# Autodesk Inventor assembly: Existing_Attic
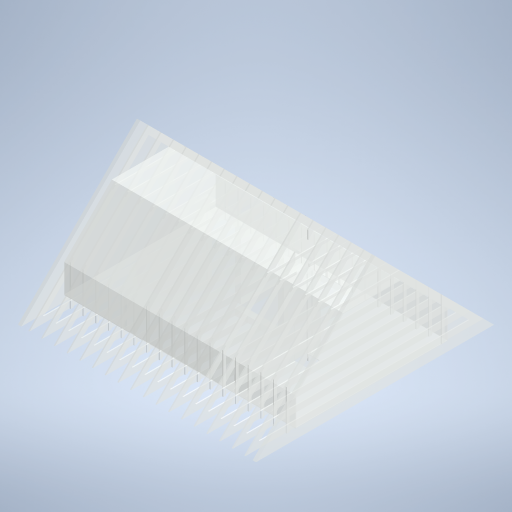
[picture p0: Inventor's stored thumbnail of the model, 512x512]
Saved by Autodesk Inventor 2024 (Build 280153000, 153)
## iProperties
Created: 2023-05-19
Part Number: Existing_Attic
Document SubType Name: Assembly
Designer: Tom
Author: Tom
## Documents named in this file (17)
- C:\Users\Tom\Documents\Tom_Levers_Public_Git_Repository\Inventor\Mobility\Attic\Existing_Attic.iam
- C:\Users\Tom\Documents\Tom_Levers_Public_Git_Repository\Inventor\Mobility\Attic\Gable.ipt
- C:\Users\Tom\Documents\Tom_Levers_Public_Git_Repository\Inventor\Mobility\Attic\Truss.ipt
- C:\Users\Tom\Documents\Tom_Levers_Public_Git_Repository\Inventor\Mobility\Attic\Sheathing.ipt
- C:\Users\Tom\Documents\Tom_Levers_Public_Git_Repository\Inventor\Mobility\Attic\Beam--7.5_x_7.5_x_46.5.ipt
- C:\Users\Tom\Documents\Tom_Levers_Public_Git_Repository\Inventor\Mobility\Attic\Second_Subfloor.ipt
- C:\Users\Tom\Documents\Tom_Levers_Public_Git_Repository\Inventor\Mobility\Attic\Knee_Wall.ipt
- C:\Users\Tom\Documents\Tom_Levers_Public_Git_Repository\Inventor\Mobility\Attic\Second_Ceiling.ipt
- C:\Users\Tom\Documents\Tom_Levers_Public_Git_Repository\Inventor\Mobility\Attic\Drywall_On_Rafters.ipt
- C:\Users\Tom\Documents\Tom_Levers_Public_Git_Repository\Inventor\Mobility\Attic\Wall_Between_Attic_Room_And_Stairwell.ipt
- C:\Users\Tom\Documents\Tom_Levers_Public_Git_Repository\Inventor\Mobility\Attic\Wall_With_Door_For_Attic_Room.ipt
- C:\Users\Tom\Documents\Tom_Levers_Public_Git_Repository\Inventor\Mobility\Attic\Wall_Between_Attic_Room_And_Landing.ipt
- C:\Users\Tom\Documents\Tom_Levers_Public_Git_Repository\Inventor\Mobility\Attic\Tar_Paper.ipt
- C:\Users\Tom\Documents\Tom_Levers_Public_Git_Repository\Inventor\Mobility\Attic\Shingles_On_Tar_Paper.ipt
- C:\Users\Tom\Documents\Tom_Levers_Public_Git_Repository\Inventor\Mobility\Attic\Ridge_Vent.ipt
- C:\Users\Tom\Documents\Tom_Levers_Public_Git_Repository\Inventor\Mobility\Attic\Shingles_On_Ridge_Vent.ipt
- C:\Users\Tom\Documents\Tom_Levers_Public_Git_Repository\Inventor\Mobility\Attic\Drywall.ipt
## Components (43 placed, 16 different names)
1. Gable:1 — Flush:1, Flush:2, Mate:1, Flush:3, Flush:4, Flush:14, Flush:15, Mate:22, Mate:47
2. Gable:2 — Flush:1, Flush:2, Mate:1, Mate:3, Flush:5, Flush:6, Flush:7, Mate:4, Flush:8, Mate:10
3. Sheathing:1 — Mate:3, Flush:5, Flush:6, Flush:23, Mate:39, Flush:24, Flush:26, Flush:29
4. Sheathing:2 — Flush:7, Mate:4, Flush:8, Mate:38, Flush:22, Flush:25, Flush:27, Flush:28, Flush:30
5. Beam--7.5_x_7.5_x_46.5:1 — Mate:5, Flush:9, Mate:6
6. Beam--7.5_x_7.5_x_46.5:2 — Flush:10, Mate:8, Mate:9
7. Second_Subfloor:1 — Mate:10, Mate:11, Mate:12, Flush:11, Mate:13, Flush:12, Mate:15, Flush:13, Mate:25, Flush:18, Mate:27, Flush:19, Mate:29, Mate:31, Mate:32, Mate:35, Mate:49
8. Knee_Wall:1 — Flush:11, Mate:13, Mate:14, Mate:19, Mate:33, Mate:36
9. Knee_Wall:2 — Flush:12, Mate:15, Mate:16, Mate:24, Mate:26
10. Second_Ceiling:1 — Mate:17, Flush:13, Flush:15, Flush:16, Flush:17, Mate:23
11. Drywall_On_Rafters:1 — Flush:16, Mate:18, Mate:19
12. Drywall_On_Rafters:2 — Flush:17, Mate:21, Mate:23
13. Drywall:1 — Mate:47, Mate:48, Mate:49
14. Wall_Between_Attic_Room_And_Stairwell:1 — Mate:24, Mate:25, Flush:18, Mate:30, Flush:21
15. Wall_Between_Attic_Room_And_Stairwell:2 — Mate:26, Mate:27, Flush:19, Mate:28, Flush:20
16. Wall_With_Door_For_Attic_Room:1 — Mate:28, Flush:20, Mate:29, Mate:50
17. Wall_With_Door_For_Attic_Room:2 — Mate:30, Flush:21, Mate:31, Mate:37
18. Wall_Between_Attic_Room_And_Landing:1 — Mate:32, Mate:33, Mate:50
19. Wall_Between_Attic_Room_And_Landing:2 — Mate:35, Mate:36, Mate:37
20. Tar_Paper:1 — Mate:38, Flush:22, Flush:23, Mate:41
21. Tar_Paper:2 — Mate:39, Flush:24, Flush:25, Mate:40
22. Shingles_On_Tar_Paper:1 — Mate:40, Flush:26, Flush:27, Mate:42
23. Shingles_On_Tar_Paper:2 — Mate:41, Flush:28, Flush:29, Mate:43
24. Ridge_Vent:1 — Mate:42, Mate:43, Flush:30, Mate:44, Mate:45, Flush:31
25. Shingles_On_Ridge_Vent:1 — Mate:44, Mate:45, Flush:31
26. Truss:1 — Flush:3, Flush:4, Mate:22
27. Truss:2 — Mate:12
28. Truss:3
29. Truss:4
30. Truss:5 — Mate:11
31. Truss:6
32. Truss:7
33. Truss:8 — Mate:6, Mate:8
34. Truss:9
35. Truss:10 — Mate:5, Flush:9, Flush:10
36. Truss:11 — Mate:9
37. Truss:12
38. Truss:13
39. Truss:14
40. Truss:15
41. Truss:16
42. Truss:17
43. Truss:18 — Mate:14, Mate:16, Mate:17, Mate:18, Mate:20, Mate:21, Mate:48
## Component patterns: (18 elements, first: Truss:1)
## Relationships (77: Mate 46, Flush 31)
- Flush:1: Gable:1 ↔ Gable:2
- Flush:2: Gable:1 ↔ Gable:2
- Mate:1 (7404.1 mm): Gable:1 ↔ Gable:2
- Flush:3: Gable:1 ↔ Truss:1
- Flush:4: Gable:1 ↔ Truss:1
- Mate:3: Gable:2 ↔ Sheathing:1
- Flush:5 (88.9 mm): Gable:2 ↔ Sheathing:1
- Flush:6: Gable:2 ↔ Sheathing:1
- Flush:7 (88.9 mm): Gable:2 ↔ Sheathing:2
- Mate:4: Gable:2 ↔ Sheathing:2
- Flush:8: Gable:2 ↔ Sheathing:2
- Mate:5: Beam--7.5_x_7.5_x_46.5:1 ↔ Truss:10
- Flush:9: Beam--7.5_x_7.5_x_46.5:1 ↔ Truss:10
- Mate:6: Beam--7.5_x_7.5_x_46.5:1 ↔ Truss:8
- Flush:10: Beam--7.5_x_7.5_x_46.5:2 ↔ Truss:10
- Mate:8: Beam--7.5_x_7.5_x_46.5:2 ↔ Truss:8
- Mate:9: Beam--7.5_x_7.5_x_46.5:2 ↔ Truss:11
- Mate:10: Gable:2 ↔ Second_Subfloor:1
- Mate:11: Second_Subfloor:1 ↔ Truss:5
- Mate:12: Second_Subfloor:1 ↔ Truss:2
- Flush:11: Second_Subfloor:1 ↔ Knee_Wall:1
- Mate:13: Second_Subfloor:1 ↔ Knee_Wall:1
- Mate:14: Knee_Wall:1 ↔ Truss:18
- Flush:12: Second_Subfloor:1 ↔ Knee_Wall:2
- Mate:15: Second_Subfloor:1 ↔ Knee_Wall:2
- Mate:16: Knee_Wall:2 ↔ Truss:18
- Mate:17: Second_Ceiling:1 ↔ Truss:18
- Flush:13: Second_Subfloor:1 ↔ Second_Ceiling:1
- Flush:14: Gable:1
- Flush:15: Gable:1 ↔ Second_Ceiling:1
- Flush:16: Second_Ceiling:1 ↔ Drywall_On_Rafters:1
- Mate:18: Drywall_On_Rafters:1 ↔ Truss:18
- Mate:19: Knee_Wall:1 ↔ Drywall_On_Rafters:1
- Mate:20: Truss:18
- Flush:17: Second_Ceiling:1 ↔ Drywall_On_Rafters:2
- Mate:21: Drywall_On_Rafters:2 ↔ Truss:18
- Mate:22 (228.6 mm): Gable:1 ↔ Truss:1
- Mate:23: Second_Ceiling:1 ↔ Drywall_On_Rafters:2
- Mate:24: Knee_Wall:2 ↔ Wall_Between_Attic_Room_And_Stairwell:1
- Mate:25: Second_Subfloor:1 ↔ Wall_Between_Attic_Room_And_Stairwell:1
- Flush:18 (4292.6 mm): Second_Subfloor:1 ↔ Wall_Between_Attic_Room_And_Stairwell:1
- Mate:26: Knee_Wall:2 ↔ Wall_Between_Attic_Room_And_Stairwell:2
- Mate:27: Second_Subfloor:1 ↔ Wall_Between_Attic_Room_And_Stairwell:2
- Flush:19 (2984.5 mm): Second_Subfloor:1 ↔ Wall_Between_Attic_Room_And_Stairwell:2
- Mate:28: Wall_Between_Attic_Room_And_Stairwell:2 ↔ Wall_With_Door_For_Attic_Room:1
- Flush:20: Wall_Between_Attic_Room_And_Stairwell:2 ↔ Wall_With_Door_For_Attic_Room:1
- Mate:29: Second_Subfloor:1 ↔ Wall_With_Door_For_Attic_Room:1
- Mate:30: Wall_Between_Attic_Room_And_Stairwell:1 ↔ Wall_With_Door_For_Attic_Room:2
- Flush:21: Wall_Between_Attic_Room_And_Stairwell:1 ↔ Wall_With_Door_For_Attic_Room:2
- Mate:31: Second_Subfloor:1 ↔ Wall_With_Door_For_Attic_Room:2
- Mate:32: Second_Subfloor:1 ↔ Wall_Between_Attic_Room_And_Landing:1
- Mate:33: Knee_Wall:1 ↔ Wall_Between_Attic_Room_And_Landing:1
- Mate:35: Second_Subfloor:1 ↔ Wall_Between_Attic_Room_And_Landing:2
- Mate:36: Knee_Wall:1 ↔ Wall_Between_Attic_Room_And_Landing:2
- Mate:37: Wall_With_Door_For_Attic_Room:2 ↔ Wall_Between_Attic_Room_And_Landing:2
- Mate:38: Sheathing:2 ↔ Tar_Paper:1
- Flush:22: Sheathing:2 ↔ Tar_Paper:1
- Flush:23: Sheathing:1 ↔ Tar_Paper:1
- Mate:39: Sheathing:1 ↔ Tar_Paper:2
- Flush:24: Sheathing:1 ↔ Tar_Paper:2
- Flush:25: Sheathing:2 ↔ Tar_Paper:2
- Mate:40: Tar_Paper:2 ↔ Shingles_On_Tar_Paper:1
- Flush:26: Sheathing:1 ↔ Shingles_On_Tar_Paper:1
- Flush:27: Sheathing:2 ↔ Shingles_On_Tar_Paper:1
- Mate:41: Tar_Paper:1 ↔ Shingles_On_Tar_Paper:2
- Flush:28: Sheathing:2 ↔ Shingles_On_Tar_Paper:2
- Flush:29: Sheathing:1 ↔ Shingles_On_Tar_Paper:2
- Mate:42: Shingles_On_Tar_Paper:1 ↔ Ridge_Vent:1
- Mate:43: Shingles_On_Tar_Paper:2 ↔ Ridge_Vent:1
- Flush:30: Sheathing:2 ↔ Ridge_Vent:1
- Mate:44: Ridge_Vent:1 ↔ Shingles_On_Ridge_Vent:1
- Mate:45: Ridge_Vent:1 ↔ Shingles_On_Ridge_Vent:1
- Flush:31: Ridge_Vent:1 ↔ Shingles_On_Ridge_Vent:1
- Mate:47: Gable:1 ↔ Drywall:1
- Mate:48: Drywall:1 ↔ Truss:18
- Mate:49: Second_Subfloor:1 ↔ Drywall:1
- Mate:50: Wall_With_Door_For_Attic_Room:1 ↔ Wall_Between_Attic_Room_And_Landing:1
